# Autodesk Inventor assembly: rs390_w_gear
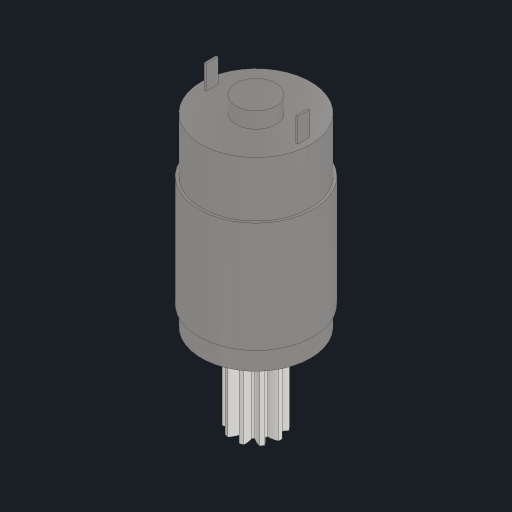
[picture p0: Inventor's stored thumbnail of the model, 512x512]
Saved by Autodesk Inventor 2023 (Build 270158000, 158)
## iProperties
Created: 2024-04-14
Part Number: rs390_w_gear
Document SubType Name: Assembly
Designer: szymo
Mass: 115.573 g
Surface Area: 72.5321 cm^2
Volume: 30.9904 cm^3
Density: 3.72931 g/cm^3
Author: szymo
## Documents named in this file (3)
- C:\zRozne\roboilo\robots\wafel\3d_parts\rs390_w_gear.iam
- C:\zRozne\roboilo\robots\wafel\3d_parts\rs390.ipt
- C:\zRozne\roboilo\robots\wafel\3d_parts\Design Accelerator\rs390_gear.iam
## Components (2 placed, 2 different names)
1. rs390:1 — Mate:1, Mate:2, Flush:1, Mate:3, Mate:4, Mate:5, Mate:6, Mate:7, Mate:8
2. Spur Gears:1 [sub-assembly] — Mate:7, Mate:8
## Relationships (9: Mate 8, Flush 1)
- Mate:1: rs390:1
- Mate:2: rs390:1
- Flush:1: rs390:1
- Mate:3: rs390:1
- Mate:4: rs390:1
- Mate:5: rs390:1
- Mate:6: rs390:1
- Mate:7: rs390:1 ↔ Spur Gears:1
- Mate:8: rs390:1 ↔ Spur Gears:1
